# Autodesk Inventor assembly: GB-assembly
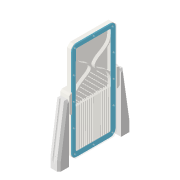
[picture p0: Inventor's stored thumbnail of the model, 180x180]
Saved by Autodesk Inventor 2020 (Build 240168000, 168)
## iProperties
Created: 2021-07-13
Part Number: GB-assembly
Document SubType Name: Assembly
Designer: Aidan Lee
Author: Aidan Lee
## Documents named in this file (6)
- C:\Users\hobly\Dropbox\Aidan Lee\Mechanics_Walk\GaltonBoard-v2\GB-assembly.iam
- C:\Users\hobly\Dropbox\Aidan Lee\Mechanics_Walk\GaltonBoard-v2\GB-glass.ipt
- C:\Users\hobly\Dropbox\Aidan Lee\Mechanics_Walk\GaltonBoard-v2\GB-hinge.ipt
- C:\Users\hobly\Dropbox\Aidan Lee\Mechanics_Walk\GaltonBoard-v2\GB-mainsection.ipt
- C:\Users\hobly\Dropbox\Aidan Lee\Mechanics_Walk\GaltonBoard-v2\GB-gasket.ipt
- C:\Users\hobly\Dropbox\Aidan Lee\Mechanics_Walk\GaltonBoard-v2\GB-stand.ipt
## Components (7 placed, 5 different names)
1. GB-glass:1 — Mate:11, Mate:12
2. GB-hinge:1 — Mate:6, Mate:7, Mate:8, Mate:16, Mate:17
3. GB-mainsection:1 — Mate:1, Mate:2, Mate:3, Mate:6, Mate:7, Mate:8, Mate:9, Mate:10
4. GB-hinge:2 — Mate:1, Mate:2, Mate:3, Mate:18, Mate:19
5. GB-gasket:1 — Mate:9, Mate:10, Mate:11, Mate:12
6. GB-stand:1 — Mate:18, Mate:19, Flush:1
7. GB-stand:2 — Mate:13, Mate:14, Mate:15, Mate:16, Mate:17, Flush:1
## Relationships (18: Mate 17, Flush 1)
- Mate:1: GB-mainsection:1 ↔ GB-hinge:2
- Mate:2: GB-mainsection:1 ↔ GB-hinge:2
- Mate:3: GB-mainsection:1 ↔ GB-hinge:2
- Mate:6: GB-hinge:1 ↔ GB-mainsection:1
- Mate:7: GB-hinge:1 ↔ GB-mainsection:1
- Mate:8: GB-hinge:1 ↔ GB-mainsection:1
- Mate:9: GB-mainsection:1 ↔ GB-gasket:1
- Mate:10: GB-mainsection:1 ↔ GB-gasket:1
- Mate:11: GB-glass:1 ↔ GB-gasket:1
- Mate:12: GB-glass:1 ↔ GB-gasket:1
- Mate:13: GB-stand:2
- Mate:14: GB-stand:2
- Mate:15: GB-stand:2
- Mate:16: GB-hinge:1 ↔ GB-stand:2
- Mate:17 (2.5 mm): GB-hinge:1 ↔ GB-stand:2
- Mate:18: GB-hinge:2 ↔ GB-stand:1
- Mate:19 (2.5 mm): GB-hinge:2 ↔ GB-stand:1
- Flush:1: GB-stand:1 ↔ GB-stand:2
